# Autodesk Inventor assembly: s-assy-shooter_unit
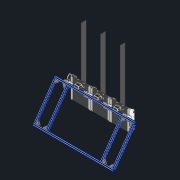
[picture p0: Inventor's stored thumbnail of the model, 180x180]
Saved by Autodesk Inventor 2022 (Build 260153000, 153)
## iProperties
Created: 2021-08-20
Part Number: s-assy-shooter_unit
Document SubType Name: Assembly
Designer: yuta0
Mass: 3751 g
Surface Area: 13652.5 cm^2
Volume: 1997.33 cm^3
Density: 1.878 g/cm^3
Author: yuta0
## Documents named in this file (14)
- C:\Users\yuta0\Desktop\catchrobo_shooter\s-assy-shooter_unit.iam
- C:\Users\yuta0\Desktop\catchrobo_shooter\s_carbon_plate1.ipt
- C:\Users\yuta0\Desktop\catchrobo_shooter\shooter_base4.ipt
- C:\Users\yuta0\Desktop\catchrobo_shooter\MF126ZZ.ipt
- C:\Users\yuta0\Desktop\catchrobo_shooter\s-assy-sorter_motor.iam
- C:\Users\yuta0\Desktop\catchrobo_shooter\s-assy-shooter_motor2.iam
- C:\Users\yuta0\Desktop\catchrobo_shooter\s-assy-sorter_plate.iam
- C:\Users\yuta0\Desktop\catchrobo_shooter\s-assy-guide_plates.iam
- C:\Users\yuta0\Desktop\catchrobo_shooter\CBSTSR3-10.ipt
- C:\Users\yuta0\Desktop\catchrobo_shooter\LBNR3.ipt
- C:\Users\yuta0\Desktop\catchrobo_shooter\CB3-15.ipt
- C:\Users\yuta0\Desktop\catchrobo_shooter\shooter_base1.ipt
- C:\Users\yuta0\Desktop\catchrobo_shooter\s-assy-frame-connector.iam
- C:\Users\yuta0\Desktop\catchrobo_shooter\s-assy-shooter_frame.iam
## Components (70 placed, 13 different names)
1. s-assy-shooter_motor2:1 [sub-assembly] — メイト:214, メイト:215, メイト:216, メイト:222
2. s-assy-guide_plates:1 [sub-assembly] — メイト:221, メイト:222, 角度:2, メイト:251, メイト:253
3. MF126ZZ:2 — メイト:55, メイト:56
4. MF126ZZ:9 — メイト:253, メイト:254
5. s-assy-shooter_frame:1 [sub-assembly] — メイト:272, メイト:273, フラッシュ:10
6. s-assy-frame-connector:3 [sub-assembly] — メイト:269, メイト:270, メイト:271, メイト:272, メイト:273
7. s-assy-frame-connector:4 [sub-assembly]
8. s-assy-frame-connector:5 [sub-assembly]
9. s-assy-frame-connector:6 [sub-assembly]
10. shooter_base1:1 — メイト:248, メイト:249, メイト:250, メイト:252, 角度:3, メイト:256, メイト:257, メイト:258, メイト:260, メイト:261
11. shooter_base4:1 — メイト:20, メイト:21, フラッシュ:6, メイト:53, メイト:54, メイト:55, メイト:56, メイト:214, メイト:215, メイト:216, メイト:226, メイト:269, メイト:270, メイト:271, フラッシュ:10
12. MF126ZZ:1 — メイト:53, メイト:54, メイト:221
13. MF126ZZ:4 — メイト:251, メイト:252
14. s_carbon_plate1:1 — メイト:20, メイト:21, フラッシュ:6, メイト:209, メイト:210, メイト:212, メイト:223, メイト:224, メイト:250
15. s-assy-sorter_motor:1 [sub-assembly] — メイト:209, メイト:210, メイト:212, メイト:217, メイト:218, 角度:1
16. s-assy-sorter_plate:1 [sub-assembly] — メイト:217, メイト:218, 角度:1
17. shooter_base1:2
18. shooter_base4:2 — メイト:255, メイト:259
19. MF126ZZ:10
20. MF126ZZ:11
21. s_carbon_plate1:2
22. s-assy-sorter_motor:2 [sub-assembly]
23. s-assy-sorter_plate:2 [sub-assembly]
24. shooter_base1:3 — メイト:254
25. shooter_base4:3
26. MF126ZZ:12
27. MF126ZZ:13
28. s_carbon_plate1:3
29. s-assy-sorter_motor:3 [sub-assembly]
30. s-assy-sorter_plate:3 [sub-assembly]
31. CB3-15:1 — メイト:245, メイト:258
32. CB3-15:2 — メイト:247, メイト:259, メイト:260
33. CB3-15:3 — メイト:243, メイト:255, メイト:261
34. CB3-15:4 — メイト:241, メイト:257
35. LBNR3:15 — メイト:241, 角度:5, 角度:6, フラッシュ:7
36. LBNR3:16 — メイト:243, 角度:6, フラッシュ:7, フラッシュ:8, メイト:256
37. LBNR3:17 — メイト:245, 角度:4, 角度:5, フラッシュ:8, フラッシュ:9
38. LBNR3:18 — メイト:247, 角度:3, 角度:4, フラッシュ:9
39. CB3-15:5
40. CB3-15:6
41. CB3-15:7
42. CB3-15:8
43. LBNR3:43
44. LBNR3:44
45. LBNR3:45
46. LBNR3:46
47. CBSTSR3-10:1 — メイト:223, メイト:224, メイト:225
48. LBNR3:1 — メイト:225, メイト:226
49. CBSTSR3-10:2
50. LBNR3:2
51. CBSTSR3-10:3 — メイト:248
52. LBNR3:3
53. CBSTSR3-10:4 — メイト:249
54. LBNR3:4
55. CBSTSR3-10:5
56. LBNR3:35
57. CBSTSR3-10:6
58. LBNR3:36
59. CBSTSR3-10:7
60. LBNR3:37
61. CBSTSR3-10:8
62. LBNR3:38
63. CBSTSR3-10:9
64. LBNR3:39
65. CBSTSR3-10:10
66. LBNR3:40
67. CBSTSR3-10:11
68. LBNR3:41
69. CBSTSR3-10:12
70. LBNR3:42
## Component patterns: (4 elements, first: s-assy-frame-connector:3), (3 elements, first: shooter_base1:1 + shooter_base4:1 + MF126ZZ:1 + MF126ZZ:4 + s_carbon_plate1:1 + s-assy-sorter_motor:1 + s-assy-sorter_plate:1), (2 elements, first: CB3-15:1 + CB3-15:2 + CB3-15:3 + CB3-15:4 + LBNR3:15 + LBNR3:16 + LBNR3:17 + LBNR3:18), (4 elements, first: CBSTSR3-10:1 + LBNR3:1), (4 elements, first: CBSTSR3-10:5 + LBNR3:35), (4 elements, first: CBSTSR3-10:9 + LBNR3:39)
## Relationships (54: Mate 43, Angle 6, Flush 5)
- 角度:1 [Angle] (0 deg): s-assy-sorter_motor:1 ↔ s-assy-sorter_plate:1
- 角度:2 [Angle] (0 deg): s-assy-guide_plates:1
- メイト:20 [Mate]: shooter_base4:1 ↔ s_carbon_plate1:1
- メイト:21 [Mate]: shooter_base4:1 ↔ s_carbon_plate1:1
- フラッシュ:6 [Flush]: shooter_base4:1 ↔ s_carbon_plate1:1
- メイト:53 [Mate]: shooter_base4:1 ↔ MF126ZZ:1
- メイト:54 [Mate]: shooter_base4:1 ↔ MF126ZZ:1
- メイト:55 [Mate]: MF126ZZ:2 ↔ shooter_base4:1
- メイト:56 [Mate]: MF126ZZ:2 ↔ shooter_base4:1
- メイト:209 [Mate]: s_carbon_plate1:1 ↔ s-assy-sorter_motor:1
- メイト:210 [Mate]: s_carbon_plate1:1 ↔ s-assy-sorter_motor:1
- メイト:212 [Mate]: s_carbon_plate1:1 ↔ s-assy-sorter_motor:1
- メイト:214 [Mate]: s-assy-shooter_motor2:1 ↔ shooter_base4:1
- メイト:215 [Mate]: s-assy-shooter_motor2:1 ↔ shooter_base4:1
- メイト:216 [Mate]: s-assy-shooter_motor2:1 ↔ shooter_base4:1
- メイト:217 [Mate]: s-assy-sorter_motor:1 ↔ s-assy-sorter_plate:1
- メイト:218 [Mate]: s-assy-sorter_motor:1 ↔ s-assy-sorter_plate:1
- メイト:221 [Mate]: s-assy-guide_plates:1 ↔ MF126ZZ:1
- メイト:222 [Mate]: s-assy-shooter_motor2:1 ↔ s-assy-guide_plates:1
- メイト:223 [Mate]: s_carbon_plate1:1 ↔ CBSTSR3-10:1
- メイト:224 [Mate]: s_carbon_plate1:1 ↔ CBSTSR3-10:1
- メイト:225 [Mate]: CBSTSR3-10:1 ↔ LBNR3:1
- メイト:226 [Mate]: shooter_base4:1 ↔ LBNR3:1
- メイト:241 [Mate]: CB3-15:4 ↔ LBNR3:15
- メイト:243 [Mate]: CB3-15:3 ↔ LBNR3:16
- メイト:245 [Mate]: CB3-15:1 ↔ LBNR3:17
- メイト:247 [Mate]: CB3-15:2 ↔ LBNR3:18
- メイト:248 [Mate]: shooter_base1:1 ↔ CBSTSR3-10:3
- メイト:249 [Mate]: shooter_base1:1 ↔ CBSTSR3-10:4
- メイト:250 [Mate]: shooter_base1:1 ↔ s_carbon_plate1:1
- メイト:251 [Mate]: s-assy-guide_plates:1 ↔ MF126ZZ:4
- メイト:252 [Mate]: shooter_base1:1 ↔ MF126ZZ:4
- メイト:253 [Mate]: s-assy-guide_plates:1 ↔ MF126ZZ:9
- メイト:254 [Mate]: MF126ZZ:9 ↔ shooter_base1:3
- 角度:3 [Angle] (0 deg): shooter_base1:1 ↔ LBNR3:18
- 角度:4 [Angle] (0 deg): LBNR3:17 ↔ LBNR3:18
- 角度:5 [Angle] (0 deg): LBNR3:15 ↔ LBNR3:17
- 角度:6 [Angle] (0 deg): LBNR3:15 ↔ LBNR3:16
- フラッシュ:7 [Flush]: LBNR3:15 ↔ LBNR3:16
- フラッシュ:8 [Flush]: LBNR3:16 ↔ LBNR3:17
- フラッシュ:9 [Flush]: LBNR3:17 ↔ LBNR3:18
- メイト:255 [Mate]: shooter_base4:2 ↔ CB3-15:3
- メイト:256 [Mate]: shooter_base1:1 ↔ LBNR3:16
- メイト:257 [Mate]: shooter_base1:1 ↔ CB3-15:4
- メイト:258 [Mate]: shooter_base1:1 ↔ CB3-15:1
- メイト:259 [Mate]: shooter_base4:2 ↔ CB3-15:2
- メイト:260 [Mate]: shooter_base1:1 ↔ CB3-15:2
- メイト:261 [Mate]: shooter_base1:1 ↔ CB3-15:3
- メイト:269 [Mate]: s-assy-frame-connector:3 ↔ shooter_base4:1
- メイト:270 [Mate]: s-assy-frame-connector:3 ↔ shooter_base4:1
- メイト:271 [Mate]: s-assy-frame-connector:3 ↔ shooter_base4:1
- メイト:272 [Mate]: s-assy-shooter_frame:1 ↔ s-assy-frame-connector:3
- メイト:273 [Mate]: s-assy-shooter_frame:1 ↔ s-assy-frame-connector:3
- フラッシュ:10 [Flush] (-110 mm): s-assy-shooter_frame:1 ↔ shooter_base4:1
